# Autodesk Inventor assembly: Assembly_my
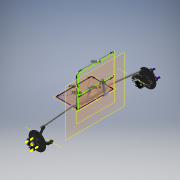
[picture p0: Inventor's stored thumbnail of the model, 180x180]
Saved by Autodesk Inventor 2019 (Build 230136000, 136)
## iProperties
Created: 2019-01-03
Part Number: Assembly_my
Document SubType Name: Assembly
Designer: keysh
Author: keysh
## Documents named in this file (4)
- F:\Assembly_my.iam
- F:\my_chassis.ipt
- F:\steering\steering assembly- kinesis.iam
- C:\Users\keysh\Downloads\brake_scaled.ipt
## Components (4 placed, 3 different names)
1. my_chassis:1 — Mate:1, Flush:3, Mate:5, Mate:7, Mate:8
2. steering assembly- kinesis:1 [sub-assembly] — Mate:1, Flush:2, Mate:2
3. brake_scaled:1 — Mate:6, Mate:7
4. brake_scaled:2 — Mate:5, Mate:6, Mate:8
## Relationships (9: Mate 6, Flush 3)
- Flush:1 (101.6 mm)
- Mate:1: my_chassis:1 ↔ steering assembly- kinesis:1
- Flush:2: steering assembly- kinesis:1
- Mate:2: steering assembly- kinesis:1
- Flush:3: my_chassis:1
- Mate:5: my_chassis:1 ↔ brake_scaled:2
- Mate:6 (150 mm): brake_scaled:1 ↔ brake_scaled:2
- Mate:7: my_chassis:1 ↔ brake_scaled:1
- Mate:8: my_chassis:1 ↔ brake_scaled:2
